# Autodesk Inventor assembly: cross_flanges
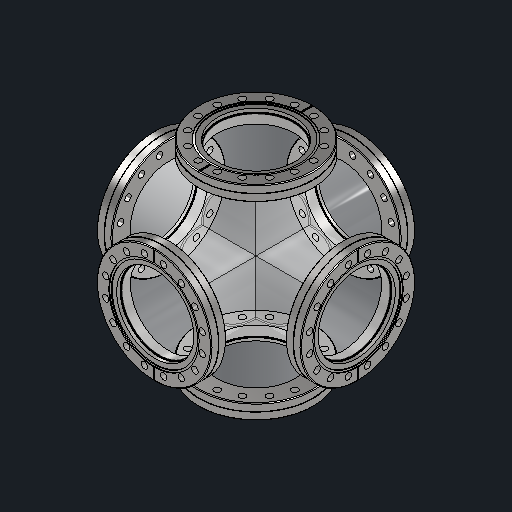
[picture p0: Inventor's stored thumbnail of the model, 512x512]
Saved by Autodesk Inventor 2026 (Build 300175050, 175E)
## iProperties
Created: 2019-06-03
Part Number: cross_flanges
Document SubType Name: Assembly
Designer: kuzmin
Mass: 9923.03 g
Surface Area: 5745.69 cm^2
Volume: 1272.81 cm^3
Density: 7.79613 g/cm^3
Author: kuzmin
## Documents named in this file (4)
- C:\Users\queez\Dropbox\Drawings\PIHTI\Plasma Vessel\Plasma-vacuum-cross\Plasma-vacuum-vessel-152IC-cross.iam
- C:\Users\queez\Dropbox\Drawings\PIHTI\Plasma Vessel\Plasma-vacuum-cross\Cross-6way-152IC.ipt
- C:\Users\queez\Dropbox\Drawings\PIHTI\Plasma Vessel\Plasma-vacuum-cross\UFC-152.ipt
- C:\Users\queez\Dropbox\Drawings\PIHTI\Plasma Vessel\Plasma-vacuum-cross\UFC.ipt
## Components (7 placed, 2 different names)
1. Cross-6way-152IC:1 — Flush:1, Mate:1, Flush:2, Rigid:1, Rigid:3, Rigid:4, Rigid:2, Rigid:5, Rigid:6
2. UFC-152:1 — Rigid:3
3. UFC-152:2 — Rigid:4
4. UFC-152:3 — Rigid:2
5. UFC-152:4 — Rigid:6
6. UFC-152:5 — Rigid:1
7. UFC-152:6 — Rigid:5
## Relationships (9: WeldJoint 6, Flush 2, Mate 1)
- Flush:1: Cross-6way-152IC:1
- Mate:1: Cross-6way-152IC:1
- Flush:2: Cross-6way-152IC:1
- Rigid:1 [WeldJoint]: Cross-6way-152IC:1 ↔ UFC-152:5
- Rigid:3 [WeldJoint]: Cross-6way-152IC:1 ↔ UFC-152:1
- Rigid:4 [WeldJoint]: Cross-6way-152IC:1 ↔ UFC-152:2
- Rigid:2 [WeldJoint]: Cross-6way-152IC:1 ↔ UFC-152:3
- Rigid:5 [WeldJoint]: Cross-6way-152IC:1 ↔ UFC-152:6
- Rigid:6 [WeldJoint]: Cross-6way-152IC:1 ↔ UFC-152:4
